# Autodesk Inventor assembly: 5 Barras Version 0
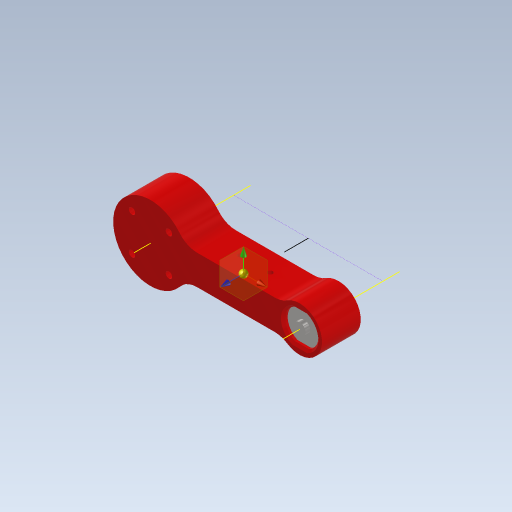
[picture p0: Inventor's stored thumbnail of the model, 512x512]
Saved by Autodesk Inventor 2024.2 (Build 282272000, 272)
## iProperties
Created: 2025-02-06
Part Number: 5 Barras Version 0
Document SubType Name: Assembly
Designer: jp.reyesf
Mass: 656.397 g
Surface Area: 470.567 cm^2
Volume: 271.333 cm^3
Author: jp.reyesf
## Documents named in this file (7)
- C:\Users\jp.reyesf\Desktop\Master-Thesis\five_bar\assets\CAD\Robot\Subassemblies\Proximal Link 1.iam
- C:\Users\jp.reyesf\Desktop\Master-Thesis\five_bar\assets\CAD\Robot\Proximal Link 2.ipt
- C:\Users\jp.reyesf\Desktop\Master-Thesis\five_bar\assets\CAD\Robot\Spacer.ipt
- C:\Users\jp.reyesf\Desktop\Master-Thesis\five_bar\assets\CAD\Robot\Bearing.ipt
- C:\Users\jp.reyesf\Desktop\Master-Thesis\five_bar\assets\CAD\Robot\separator.ipt
- C:\Users\jp.reyesf\Desktop\Master-Thesis\five_bar\assets\CAD\Robot\rod.ipt
- C:\Users\jp.reyesf\Desktop\Master-Thesis\five_bar\assets\CAD\Robot\Subassemblies\DummyBar.ipt
## Components (7 placed, 6 different names)
1. Proximal Link 2:1 — Mate:35, Flush:9, Mate:54, Flush:10, Angle:1, Mate:58, Flush:11, Flush:12, Mate:60, Mate:61
2. separator:2 — Mate:56, Mate:58
3. Spacer:2 — Mate:35
4. Bearing:4 — Mate:59
5. Bearing:5 — Flush:12
6. rod:3 — Flush:9, Mate:54, Mate:56
7. DummyBar:1 — Mate:59, Flush:11
## Relationships (16: Mate 11, Flush 4, Angle 1)
- [Mate]: Spacer:2 ↔ Bearing:4
- [Mate]: Spacer:2 ↔ Bearing:5
- [Mate]: Spacer:2 ↔ Bearing:4
- [Mate]: Spacer:2 ↔ Bearing:5
- Mate:35: Proximal Link 2:1 ↔ Spacer:2
- Flush:9: Proximal Link 2:1 ↔ rod:3
- Mate:54: Proximal Link 2:1 ↔ rod:3
- Mate:56: separator:2 ↔ rod:3
- Flush:10: Proximal Link 2:1
- Angle:1 (180 deg): Proximal Link 2:1
- Mate:58: Proximal Link 2:1 ↔ separator:2
- Mate:59: Bearing:4 ↔ DummyBar:1
- Flush:11: Proximal Link 2:1 ↔ DummyBar:1
- Flush:12: Proximal Link 2:1 ↔ Bearing:5
- Mate:60: Proximal Link 2:1
- Mate:61: Proximal Link 2:1
## Named parameters: d18_d14 = 0 mm, d19_d15 = 0 mm, d20_d16 = 0 mm, d21_d17 = 0 mm
